# Autodesk Inventor assembly: main
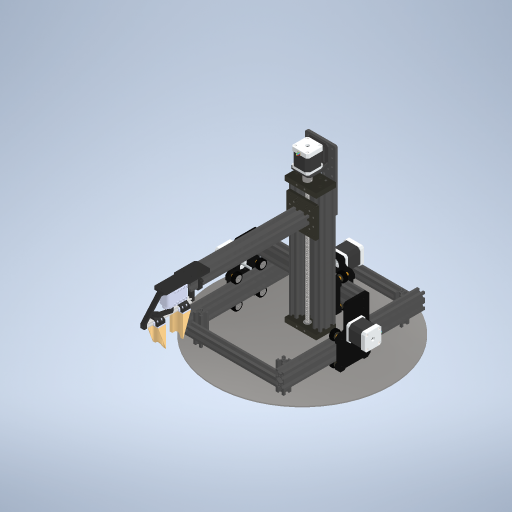
[picture p0: Inventor's stored thumbnail of the model, 512x512]
Saved by Autodesk Inventor 2024.2 (Build 282272000, 272)
## iProperties
Created: 2024-08-26
Part Number: main
Document SubType Name: Assembly
Designer: Admin
Author: Admin
## Documents named in this file (8)
- C:\Users\Admin\Documents\GitHub\RobotCartesiano\DiseñoBrazo\Assemblies\main.iam
- C:\Users\Admin\Documents\GitHub\RobotCartesiano\DiseñoBrazo\Assemblies\AxisX.iam
- C:\Users\Admin\Documents\GitHub\RobotCartesiano\DiseñoBrazo\AuxiliarPieces\FestinoRobot\AluminumBase.ipt
- C:\Users\Admin\Documents\GitHub\RobotCartesiano\DiseñoBrazo\Assemblies\AxisY.iam
- C:\Users\Admin\Documents\GitHub\RobotCartesiano\DiseñoBrazo\Assemblies\AxisZ.iam
- C:\Users\Admin\Documents\GitHub\RobotCartesiano\DiseñoBrazo\Assemblies\MovingPlate.iam
- C:\Users\Admin\Documents\GitHub\RobotCartesiano\DiseñoBrazo\Assemblies\FinalClaw\Claw.iam
- C:\Users\Admin\Documents\GitHub\RobotCartesiano\DiseñoBrazo\Assemblies\FinalClaw\SoporteY\SoporteY.ipt
## Components (7 placed, 7 different names)
1. AluminumBase:1 — Mate:1
2. AxisX:1 [sub-assembly] — Mate:1, Tangent:1, Tangent:2, Tangent:3
3. AxisY:1 [sub-assembly] — Tangent:1, Tangent:2, Tangent:3, Tangent:4, Tangent:5, Tangent:6, Tangent:7
4. AxisZ:1 [sub-assembly] — Tangent:4, Tangent:5, Tangent:6, Tangent:7, Mate:2
5. MovingPlate:1 [sub-assembly] — Mate:2, Mate:3, Flush:1, Mate:4, Mate:5, Mate:6
6. Claw:1 [sub-assembly] — Mate:3, Flush:1, Mate:4, Mate:7
7. SoporteY:1 — Mate:5, Mate:6, Mate:7
## Relationships (15: Mate 7, Tangent 7, Flush 1)
- Mate:1: AluminumBase:1 ↔ AxisX:1
- Tangent:1: AxisX:1 ↔ AxisY:1
- Tangent:2: AxisX:1 ↔ AxisY:1
- Tangent:3: AxisX:1 ↔ AxisY:1
- Tangent:4: AxisY:1 ↔ AxisZ:1
- Tangent:5: AxisY:1 ↔ AxisZ:1
- Tangent:6: AxisY:1 ↔ AxisZ:1
- Tangent:7: AxisY:1 ↔ AxisZ:1
- Mate:2: AxisZ:1 ↔ MovingPlate:1
- Mate:3: MovingPlate:1 ↔ Claw:1
- Flush:1: MovingPlate:1 ↔ Claw:1
- Mate:4: MovingPlate:1 ↔ Claw:1
- Mate:5: MovingPlate:1 ↔ SoporteY:1
- Mate:6: MovingPlate:1 ↔ SoporteY:1
- Mate:7: Claw:1 ↔ SoporteY:1
